# Autodesk Inventor assembly: LauncherReassembly
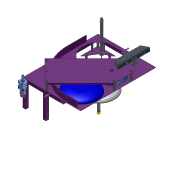
[picture p0: Inventor's stored thumbnail of the model, 180x180]
Saved by Autodesk Inventor 2012 (Build 160160000, 160)
## iProperties
Created: 2013-01-22
Part Number: LauncherReassembly
Document SubType Name: Assembly
Designer: JesseK
Mass: 5443.33 g
Surface Area: 30706.7 cm^2
Volume: 4981.79 cm^3
Density: 1.09265 g/cm^3
Author: JesseK
## Documents named in this file (13)
- Z:\UserData\Documents\Inventor\team1885frc\Robot2013\LauncherRearrange\LauncherReassembly.iam
- Z:\UserData\Documents\Inventor\team1885frc\Robot2013\LauncherRearrange\LauncherFrame.iam
- Z:\UserData\Documents\Inventor\team1885frc\Robot2013\Launcher\90 degree curved shooter v1.iam
- Z:\UserData\Documents\Inventor\team1885frc\Robot2013\LauncherRearrange\LauncherRotationAxle.ipt
- Z:\UserData\Documents\Inventor\team1885frc\Robot2013\Hopper\CylinderOffsetPlate.ipt
- Z:\UserData\Documents\Inventor\team1885frc\Pneumatics\047-DXP_7inStrokex075Bore\047_DXP_R_D_129__F_D_166_3_.iam
- Z:\UserData\Documents\Inventor\team1885frc\Robot2013\LauncherRearrange\HopperPlateOffset.ipt
- Z:\UserData\Documents\Inventor\team1885frc\Pneumatics\047-DXP_7inStrokex075Bore\D_9.ipt
- Z:\UserData\Documents\Inventor\team1885frc\Robot2013\Hopper\HopperAssembly.iam
- Z:\UserData\Documents\Inventor\team1885frc\VEXPro\VersaPlanetary Gearbox\217-2625 with AM-9015.20121205\217-2625 with AM-9015.20121205.iam
- Z:\UserData\Documents\Inventor\team1885frc\Kinect\kinect assembly.iam
- Z:\UserData\Documents\Inventor\team1885frc\Robot2013\LauncherRearrange\HopperGuide2.ipt
- Z:\UserData\Documents\Inventor\team1885frc\Hardware\Bolts\Bolt_0.25_20_0.75len_SocketHead.ipt
## Components (21 placed, 12 different names)
1. LauncherFrame:1 [sub-assembly] — Mate:1, Flush:1, Mate:2, Mate:3, Mate:4, Flush:2, Flush:3, Flush:4, Mate:6, Mate:15, Mate:29, Flush:5
2. 90 degree curved shooter v1:1 [sub-assembly] — Mate:1, Flush:1, Mate:2, Mate:30, Flush:6
3. LauncherRotationAxle:1 — Mate:3, Flush:3
4. LauncherRotationAxle:2 — Mate:4, Flush:2
5. CylinderOffsetPlate:1 — Flush:4, Mate:6, Mate:7, Mate:8, Mate:9, Mate:10, Mate:11, Mate:12, Mate:13, Mate:14, Mate:16, Mate:32, Mate:33, Mate:34, Mate:35, Mate:36, Mate:37, Mate:38, Mate:39, Mate:40, Mate:41, Mate:42, Mate:43, Mate:44, Mate:45
6. 047-DXP:1 [sub-assembly] — Mate:7, Mate:8, Mate:17, Mate:22, Mate:23
7. HopperPlateOffset:1 — Mate:9, Mate:14, Mate:15
8. HopperPlateOffset:2 — Mate:10, Mate:13
9. HopperPlateOffset:3 — Mate:11, Mate:12
10. D-9:1 — Mate:16, Mate:17
11. CylinderOffsetPlate:2 — Mate:22, Mate:23, Mate:25, Mate:26, Mate:31
12. HopperAssembly:1 [sub-assembly] — Mate:25, Mate:26
13. 217-2625 with AM-9015.20121205:1 [sub-assembly] — Mate:29, Flush:5
14. kinect assembly:1 [sub-assembly] — Mate:30, Flush:6
15. HopperGuide2:1 — Mate:31, Mate:32, Mate:35
16. HopperGuide2:2 — Mate:33, Mate:34
17. Bolt_0.25_20_0.75len_SocketHead:1 — Mate:36, Mate:39
18. Bolt_0.25_20_0.75len_SocketHead:2 — Mate:37, Mate:38
19. Bolt_0.25_20_0.75len_SocketHead:3 — Mate:42, Mate:45
20. Bolt_0.25_20_0.75len_SocketHead:4 — Mate:41, Mate:44
21. Bolt_0.25_20_0.75len_SocketHead:5 — Mate:40, Mate:43
## Relationships (43: Mate 37, Flush 6)
- Mate:1: LauncherFrame:1 ↔ 90 degree curved shooter v1:1
- Flush:1: LauncherFrame:1 ↔ 90 degree curved shooter v1:1
- Mate:2: LauncherFrame:1 ↔ 90 degree curved shooter v1:1
- Mate:3: LauncherFrame:1 ↔ LauncherRotationAxle:1
- Mate:4: LauncherFrame:1 ↔ LauncherRotationAxle:2
- Flush:2: LauncherFrame:1 ↔ LauncherRotationAxle:2
- Flush:3: LauncherFrame:1 ↔ LauncherRotationAxle:1
- Flush:4: LauncherFrame:1 ↔ CylinderOffsetPlate:1
- Mate:6: LauncherFrame:1 ↔ CylinderOffsetPlate:1
- Mate:7: CylinderOffsetPlate:1 ↔ 047-DXP:1
- Mate:8: CylinderOffsetPlate:1 ↔ 047-DXP:1
- Mate:9: CylinderOffsetPlate:1 ↔ HopperPlateOffset:1
- Mate:10: CylinderOffsetPlate:1 ↔ HopperPlateOffset:2
- Mate:11: CylinderOffsetPlate:1 ↔ HopperPlateOffset:3
- Mate:12: CylinderOffsetPlate:1 ↔ HopperPlateOffset:3
- Mate:13: CylinderOffsetPlate:1 ↔ HopperPlateOffset:2
- Mate:14: CylinderOffsetPlate:1 ↔ HopperPlateOffset:1
- Mate:15: LauncherFrame:1 ↔ HopperPlateOffset:1
- Mate:16: CylinderOffsetPlate:1 ↔ D-9:1
- Mate:17: 047-DXP:1 ↔ D-9:1
- Mate:22: 047-DXP:1 ↔ CylinderOffsetPlate:2
- Mate:23: 047-DXP:1 ↔ CylinderOffsetPlate:2
- Mate:25 (6.35 mm): CylinderOffsetPlate:2 ↔ HopperAssembly:1
- Mate:26: CylinderOffsetPlate:2 ↔ HopperAssembly:1
- Mate:29: LauncherFrame:1 ↔ 217-2625 with AM-9015.20121205:1
- Flush:5: LauncherFrame:1 ↔ 217-2625 with AM-9015.20121205:1
- Mate:30: 90 degree curved shooter v1:1 ↔ kinect assembly:1
- Flush:6 (76.2 mm): 90 degree curved shooter v1:1 ↔ kinect assembly:1
- Mate:31: CylinderOffsetPlate:2 ↔ HopperGuide2:1
- Mate:32: CylinderOffsetPlate:1 ↔ HopperGuide2:1
- Mate:33: CylinderOffsetPlate:1 ↔ HopperGuide2:2
- Mate:34: CylinderOffsetPlate:1 ↔ HopperGuide2:2
- Mate:35: CylinderOffsetPlate:1 ↔ HopperGuide2:1
- Mate:36: CylinderOffsetPlate:1 ↔ Bolt_0.25_20_0.75len_SocketHead:1
- Mate:37: CylinderOffsetPlate:1 ↔ Bolt_0.25_20_0.75len_SocketHead:2
- Mate:38: CylinderOffsetPlate:1 ↔ Bolt_0.25_20_0.75len_SocketHead:2
- Mate:39: CylinderOffsetPlate:1 ↔ Bolt_0.25_20_0.75len_SocketHead:1
- Mate:40: CylinderOffsetPlate:1 ↔ Bolt_0.25_20_0.75len_SocketHead:5
- Mate:41: CylinderOffsetPlate:1 ↔ Bolt_0.25_20_0.75len_SocketHead:4
- Mate:42: CylinderOffsetPlate:1 ↔ Bolt_0.25_20_0.75len_SocketHead:3
- Mate:43: CylinderOffsetPlate:1 ↔ Bolt_0.25_20_0.75len_SocketHead:5
- Mate:44: CylinderOffsetPlate:1 ↔ Bolt_0.25_20_0.75len_SocketHead:4
- Mate:45: CylinderOffsetPlate:1 ↔ Bolt_0.25_20_0.75len_SocketHead:3
